# Autodesk Inventor assembly: Reality
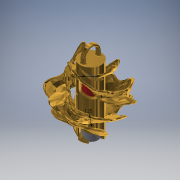
[picture p0: Inventor's stored thumbnail of the model, 180x180]
Saved by Autodesk Inventor 2019 (Build 230136000, 136)
## iProperties
Created: 2019-05-18
Part Number: Reality
Document SubType Name: Assembly
Designer: Jorian Brusind
Author: Jorian Brusind
## Documents named in this file (4)
- C:\Users\Jorian Brusind\Documents\GitHub\PersonalProjects\Inventor Projects\Infinity\Reality.iam
- C:\Users\Jorian Brusind\Documents\GitHub\PersonalProjects\Inventor Projects\Infinity\Waves.ipt
- C:\Users\Jorian Brusind\Documents\GitHub\PersonalProjects\Inventor Projects\Infinity\Red.ipt
- C:\Users\Jorian Brusind\Documents\GitHub\PersonalProjects\Inventor Projects\Infinity\EndCap.ipt
## Components (4 placed, 3 different names)
1. Waves:1 — Mate:1, Mate:2, Mate:3, Mate:4, Flush:1
2. Red:1 — Mate:1, Mate:5
3. EndCap:1 — Mate:4, Flush:1, Mate:5
4. EndCap:2 — Mate:2, Mate:3
## Relationships (6: Mate 5, Flush 1)
- Mate:1: Waves:1 ↔ Red:1
- Mate:2: Waves:1 ↔ EndCap:2
- Mate:3: Waves:1 ↔ EndCap:2
- Mate:4: Waves:1 ↔ EndCap:1
- Flush:1: Waves:1 ↔ EndCap:1
- Mate:5: Red:1 ↔ EndCap:1
